# Autodesk Inventor assembly: REV-41-1097
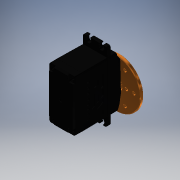
[picture p0: Inventor's stored thumbnail of the model, 180x180]
Saved by Autodesk Inventor 2018 (Build 220112000, 112)
## iProperties
Created: 2015-09-14
Part Number: REV-41-1097
Description: STEP AP203
Document SubType Name: Assembly
Designer: S-2512711
Sending System: SolidWorks 2014
Preprocessor: SwSTEP 2.0
Title: REV-41-1097.STEP
Revision Number: ANY
## Documents named in this file (7)
- C:\Users\maste\OneDrive\Documents\GitHub\2020CAD\Control panel spinny boi\Part Files\REV-41-1097.iam
- C:\Users\maste\OneDrive\Documents\GitHub\2020CAD\Control panel spinny boi\Part Files\A.ipt
- C:\Users\maste\OneDrive\Documents\GitHub\2020CAD\Control panel spinny boi\Part Files\E.ipt
- C:\Users\maste\OneDrive\Documents\GitHub\2020CAD\Control panel spinny boi\Part Files\C.ipt
- C:\Users\maste\OneDrive\Documents\GitHub\2020CAD\Control panel spinny boi\Part Files\B.ipt
- C:\Users\maste\OneDrive\Documents\GitHub\2020CAD\Control panel spinny boi\Part Files\D.ipt
- C:\Users\maste\OneDrive\Documents\GitHub\2020CAD\Control panel spinny boi\Part Files\REV-41-1363.ipt
## Components (6 placed, 6 different names)
1. A_1
2. E_2
3. C_3 — Mate:2, Rotation:1
4. B_4
5. D_5 — Mate:1
6. REV-41-1363:1 — Mate:1, Mate:2, Rotation:1
## Relationships (3: Mate 2, RelateRotation 1)
- Mate:1: D_5 ↔ REV-41-1363:1
- Mate:2: C_3 ↔ REV-41-1363:1
- Rotation:1 [RelateRotation] (1 ul): C_3 ↔ REV-41-1363:1
